# Autodesk Inventor assembly: LCD+Case
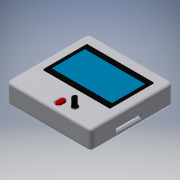
[picture p0: Inventor's stored thumbnail of the model, 180x180]
Saved by Autodesk Inventor 2016 (Build 200138000, 138)
## iProperties
Created: 2015-04-16
Part Number: LCD+Case
Document SubType Name: Assembly
Designer: Jack
Author: Jack
Title: Graphic LCD Knockoff + Case
## Documents named in this file (7)
- C:\Users\Jack\ownCloud\Projects\CrossBot\InventorModel\Enclosure\LCDCase\LCD+Case.iam
- C:\Users\Jack\ownCloud\Projects\CrossBot\InventorModel\Electronics\LCD\GLCDKnockoff.ipt
- C:\Users\Jack\ownCloud\Projects\CrossBot\InventorModel\Enclosure\LCDCase\LCDDerivativeBottom1.ipt
- C:\Users\Jack\ownCloud\Projects\CrossBot\InventorModel\Enclosure\LCDCase\LCDDerivativeTop1.ipt
- C:\Users\Jack\ownCloud\Projects\CrossBot\InventorModel\Enclosure\LCDCase\LCDButton.ipt
- C:\Users\Jack\ownCloud\Projects\CrossBot\InventorModel\Hardware\Nuts\Nut3.ipt
- C:\Users\Jack\ownCloud\Projects\CrossBot\InventorModel\Hardware\Bolts\SHCS\SHCS3\SHCS3x16.ipt
## Components (12 placed, 6 different names)
1. GLCDKnockoff:1 — Mate:3, Mate:4, Mate:5, Mate:6, Mate:11, Mate:12, Mate:13, Mate:17, Mate:23
2. LCDDerivativeBottom1:1 — Mate:11, Mate:12, Mate:13, Mate:23, Mate:32, Mate:33, Mate:34, Mate:35, Mate:36, Mate:37, Mate:38, Mate:39
3. LCDDerivativeTop1:1 — Mate:3, Mate:4, Mate:5, Mate:6, Mate:14, Mate:17, Mate:18, Angle:1, Mate:24, Mate:25, Mate:26, Mate:27, Mate:28, Mate:29, Mate:30, Mate:31, Angle:2, Angle:3, Angle:4, Angle:5
4. LCDButton:1 — Mate:14, Mate:18, Angle:1
5. Nut3:1 — Mate:26, Mate:29, Angle:5
6. Nut3:2 — Mate:24, Mate:30, Angle:3
7. Nut3:3 — Mate:25, Mate:31, Angle:2
8. Nut3:4 — Mate:27, Mate:28, Angle:4
9. SHCS3x16:1 — Mate:34, Mate:39
10. SHCS3x16:2 — Mate:36, Mate:37
11. SHCS3x16:3 — Mate:35, Mate:38
12. SHCS3x16:4 — Mate:32, Mate:33
## Relationships (32: Mate 27, Angle 5)
- Mate:3: GLCDKnockoff:1 ↔ LCDDerivativeTop1:1
- Mate:4: GLCDKnockoff:1 ↔ LCDDerivativeTop1:1
- Mate:5: GLCDKnockoff:1 ↔ LCDDerivativeTop1:1
- Mate:6: GLCDKnockoff:1 ↔ LCDDerivativeTop1:1
- Mate:11: GLCDKnockoff:1 ↔ LCDDerivativeBottom1:1
- Mate:12: GLCDKnockoff:1 ↔ LCDDerivativeBottom1:1
- Mate:13: GLCDKnockoff:1 ↔ LCDDerivativeBottom1:1
- Mate:14: LCDDerivativeTop1:1 ↔ LCDButton:1
- Mate:17: GLCDKnockoff:1 ↔ LCDDerivativeTop1:1
- Mate:18: LCDDerivativeTop1:1 ↔ LCDButton:1
- Mate:23: GLCDKnockoff:1 ↔ LCDDerivativeBottom1:1
- Angle:1 (180 deg): LCDDerivativeTop1:1 ↔ LCDButton:1
- Mate:24: LCDDerivativeTop1:1 ↔ Nut3:2
- Mate:25: LCDDerivativeTop1:1 ↔ Nut3:3
- Mate:26: LCDDerivativeTop1:1 ↔ Nut3:1
- Mate:27: LCDDerivativeTop1:1 ↔ Nut3:4
- Mate:28: LCDDerivativeTop1:1 ↔ Nut3:4
- Mate:29: LCDDerivativeTop1:1 ↔ Nut3:1
- Mate:30: LCDDerivativeTop1:1 ↔ Nut3:2
- Mate:31: LCDDerivativeTop1:1 ↔ Nut3:3
- Angle:2 (0 deg): LCDDerivativeTop1:1 ↔ Nut3:3
- Angle:3 (0 deg): LCDDerivativeTop1:1 ↔ Nut3:2
- Angle:4 (0 deg): LCDDerivativeTop1:1 ↔ Nut3:4
- Angle:5 (0 deg): LCDDerivativeTop1:1 ↔ Nut3:1
- Mate:32: LCDDerivativeBottom1:1 ↔ SHCS3x16:4
- Mate:33: LCDDerivativeBottom1:1 ↔ SHCS3x16:4
- Mate:34: LCDDerivativeBottom1:1 ↔ SHCS3x16:1
- Mate:35: LCDDerivativeBottom1:1 ↔ SHCS3x16:3
- Mate:36: LCDDerivativeBottom1:1 ↔ SHCS3x16:2
- Mate:37: LCDDerivativeBottom1:1 ↔ SHCS3x16:2
- Mate:38: LCDDerivativeBottom1:1 ↔ SHCS3x16:3
- Mate:39: LCDDerivativeBottom1:1 ↔ SHCS3x16:1
